# Autodesk Inventor assembly: BOB Assembly
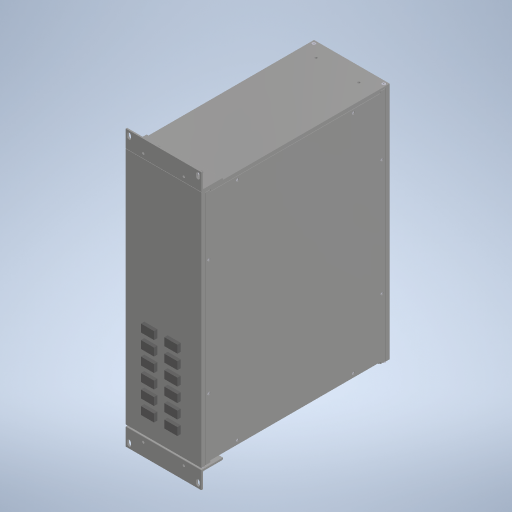
[picture p0: Inventor's stored thumbnail of the model, 512x512]
Saved by Autodesk Inventor 2023 (Build 270158000, 158)
## iProperties
Created: 2024-02-19
Part Number: BOB Assembly
Document SubType Name: Assembly
Designer: Matthijs Rog
Author: Matthijs Rog
## Documents named in this file (5)
- C:\PhD\Teslatron\Teslatron_BOB\InventorFiles\BOB Assembly.iam
- C:\PhD\Teslatron\Teslatron_BOB\InventorFiles\RM3U1913SBK.iam
- C:\PhD\Teslatron\Teslatron_BOB\InventorFiles\GND_Switch_Board.iam
- C:\PhD\Teslatron\Teslatron_BOB\InventorFiles\SMA_Feedthrough_Board.iam
- C:\PhD\Teslatron\Teslatron_BOB\InventorFiles\Download_STEP_709905691 (rev1).ipt
## Components (9 placed, 4 different names)
1. RM3U1913SBK:1 [sub-assembly]
2. GND_Switch_Board:1 [sub-assembly]
3. SMA_Feedthrough_Board:1 [sub-assembly] — Rotational:6, Rotational:7
4. SMA_Feedthrough_Board:2 [sub-assembly] — Rotational:1, Rotational:2, Rotational:3, Rotational:4, Rotational:5
5. Download_STEP_709905691 (rev1):1 — Rotational:1
6. Download_STEP_709905691 (rev1):2 — Rotational:4
7. Download_STEP_709905691 (rev1):3 — Rotational:5, Rotational:6
8. Download_STEP_709905691 (rev1):5 — Rotational:2
9. Download_STEP_709905691 (rev1):6 — Rotational:3, Rotational:7
## Relationships (7: RevoluteJoint 7)
- Rotational:1 [RevoluteJoint]: SMA_Feedthrough_Board:2 ↔ Download_STEP_709905691 (rev1):1
- Rotational:2 [RevoluteJoint]: SMA_Feedthrough_Board:2 ↔ Download_STEP_709905691 (rev1):5
- Rotational:3 [RevoluteJoint]: SMA_Feedthrough_Board:2 ↔ Download_STEP_709905691 (rev1):6
- Rotational:4 [RevoluteJoint]: SMA_Feedthrough_Board:2 ↔ Download_STEP_709905691 (rev1):2
- Rotational:5 [RevoluteJoint]: SMA_Feedthrough_Board:2 ↔ Download_STEP_709905691 (rev1):3
- Rotational:6 [RevoluteJoint]: SMA_Feedthrough_Board:1 ↔ Download_STEP_709905691 (rev1):3
- Rotational:7 [RevoluteJoint]: SMA_Feedthrough_Board:1 ↔ Download_STEP_709905691 (rev1):6
